# Autodesk Inventor assembly: Flywheel Axle Assembly v11
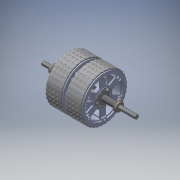
[picture p0: Inventor's stored thumbnail of the model, 180x180]
Saved by Autodesk Inventor 2018 (Build 220112000, 112)
## iProperties
Created: 2020-01-29
Part Number: Flywheel Axle Assembly v11
Document SubType Name: Assembly
Designer: s-2512711
Author: s-2512711
## Documents named in this file (10)
- \\studenthome\students\S-2512711\GitHub\2020CAD\New Gabriel Shooter\ACTUAL ASSEMBLY FILES\Flywheel Axle Assembly v11.iam
- \\studenthome\students\S-2512711\GitHub\2020CAD\New Gabriel Shooter\ACTUAL ASSEMBLY FILES\am-2986 FR8ZZ Hex Bearing v1.ipt
- \\studenthome\students\S-2512711\GitHub\2020CAD\New Gabriel Shooter\ACTUAL ASSEMBLY FILES\6_Traction_Tire_mounted_on_6_Traction_Wheel v1.iam
- \\studenthome\students\S-2512711\GitHub\2020CAD\New Gabriel Shooter\ACTUAL ASSEMBLY FILES\6_Traction_Tire_mounted_on_6_Traction_Wheel v1_1.iam
- \\studenthome\students\S-2512711\GitHub\2020CAD\New Gabriel Shooter\ACTUAL ASSEMBLY FILES\1_2_Hex_Bore_Aluminum_VersaHub_217-2592 v1.ipt
- \\studenthome\students\S-2512711\GitHub\2020CAD\New Gabriel Shooter\ACTUAL ASSEMBLY FILES\1_2_Acetal_Spacer_-_1_2_Hex_217-3261 v1.ipt
- \\studenthome\students\S-2512711\GitHub\2020CAD\New Gabriel Shooter\ACTUAL ASSEMBLY FILES\1_16_Acetal_Spacer_-_1_2_Hex_217-3257 v1.ipt
- \\studenthome\students\S-2512711\GitHub\2020CAD\New Gabriel Shooter\ACTUAL ASSEMBLY FILES\1_Acetal_Spacer_-_1_2_Hex_217-3263 v1.ipt
- \\studenthome\students\S-2512711\GitHub\2020CAD\New Gabriel Shooter\ACTUAL ASSEMBLY FILES\1_4_Acetal_Spacer_-_1_2_Hex_217-3259 v1.ipt
- \\studenthome\students\S-2512711\GitHub\2020CAD\New Gabriel Shooter\ACTUAL ASSEMBLY FILES\Flywheel Axle Assembly v11.ipt
## Components (18 placed, 8 different names)
1. am-2986 FR8ZZ Hex Bearing v1:1 — Mate:19, Mate:20, Mate:21
2. am-2986 FR8ZZ Hex Bearing v1:2 — Mate:1, Mate:2, Mate:3
3. 6_Traction_Tire_mounted_on_6_Traction_Wheel v1:1 [sub-assembly] — Mate:26, Mate:27, Mate:28, Mate:29, Mate:30, Mate:31
4. 6_Traction_Tire_mounted_on_6_Traction_Wheel v1:2 [sub-assembly] — Mate:10, Mate:11, Mate:12, Mate:13, Mate:14, Mate:15
5. 1_2_Hex_Bore_Aluminum_VersaHub_217-2592 v1:1 — Mate:25, Mate:26, Mate:27, Mate:28
6. 1_2_Hex_Bore_Aluminum_VersaHub_217-2592 v1:2 — Mate:29, Mate:30, Mate:31, Mate:32
7. 1_2_Hex_Bore_Aluminum_VersaHub_217-2592 v1:3 — Mate:13, Mate:14, Mate:15, Mate:18
8. 1_2_Hex_Bore_Aluminum_VersaHub_217-2592 v1:4 — Mate:7, Mate:8, Mate:9, Mate:10, Mate:11, Mate:12
9. 1_2_Acetal_Spacer_-_1_2_Hex_217-3261 v1:1 — Mate:16, Mate:17, Mate:18, Mate:32
10. 1_2_Acetal_Spacer_-_1_2_Hex_217-3261 v1:2 — Mate:23, Mate:24
11. 1_2_Acetal_Spacer_-_1_2_Hex_217-3261 v1:3 — Mate:5, Mate:6
12. 1_16_Acetal_Spacer_-_1_2_Hex_217-3257 v1:1 — Mate:3, Mate:4
13. 1_16_Acetal_Spacer_-_1_2_Hex_217-3257 v1:2 — Mate:21, Mate:22
14. 1_Acetal_Spacer_-_1_2_Hex_217-3263 v1:1 — Mate:6, Mate:7
15. 1_Acetal_Spacer_-_1_2_Hex_217-3263 v1:2 — Mate:24, Mate:25
16. 1_4_Acetal_Spacer_-_1_2_Hex_217-3259 v1:1 — Mate:22, Mate:23
17. 1_4_Acetal_Spacer_-_1_2_Hex_217-3259 v1:2 — Mate:4, Mate:5
18. Flywheel Axle Assembly v11 — Mate:1, Mate:2, Mate:8, Mate:9, Mate:16, Mate:17, Mate:19, Mate:20
## Relationships (32: Mate 32)
- Mate:1: am-2986 FR8ZZ Hex Bearing v1:2 ↔ Flywheel Axle Assembly v11
- Mate:2: am-2986 FR8ZZ Hex Bearing v1:2 ↔ Flywheel Axle Assembly v11
- Mate:3: am-2986 FR8ZZ Hex Bearing v1:2 ↔ 1_16_Acetal_Spacer_-_1_2_Hex_217-3257 v1:1
- Mate:4: 1_16_Acetal_Spacer_-_1_2_Hex_217-3257 v1:1 ↔ 1_4_Acetal_Spacer_-_1_2_Hex_217-3259 v1:2
- Mate:5: 1_2_Acetal_Spacer_-_1_2_Hex_217-3261 v1:3 ↔ 1_4_Acetal_Spacer_-_1_2_Hex_217-3259 v1:2
- Mate:6: 1_2_Acetal_Spacer_-_1_2_Hex_217-3261 v1:3 ↔ 1_Acetal_Spacer_-_1_2_Hex_217-3263 v1:1
- Mate:7: 1_2_Hex_Bore_Aluminum_VersaHub_217-2592 v1:4 ↔ 1_Acetal_Spacer_-_1_2_Hex_217-3263 v1:1
- Mate:8: 1_2_Hex_Bore_Aluminum_VersaHub_217-2592 v1:4 ↔ Flywheel Axle Assembly v11
- Mate:9: 1_2_Hex_Bore_Aluminum_VersaHub_217-2592 v1:4 ↔ Flywheel Axle Assembly v11
- Mate:10: 6_Traction_Tire_mounted_on_6_Traction_Wheel v1:2 ↔ 1_2_Hex_Bore_Aluminum_VersaHub_217-2592 v1:4
- Mate:11: 6_Traction_Tire_mounted_on_6_Traction_Wheel v1:2 ↔ 1_2_Hex_Bore_Aluminum_VersaHub_217-2592 v1:4
- Mate:12: 6_Traction_Tire_mounted_on_6_Traction_Wheel v1:2 ↔ 1_2_Hex_Bore_Aluminum_VersaHub_217-2592 v1:4
- Mate:13: 6_Traction_Tire_mounted_on_6_Traction_Wheel v1:2 ↔ 1_2_Hex_Bore_Aluminum_VersaHub_217-2592 v1:3
- Mate:14: 6_Traction_Tire_mounted_on_6_Traction_Wheel v1:2 ↔ 1_2_Hex_Bore_Aluminum_VersaHub_217-2592 v1:3
- Mate:15: 6_Traction_Tire_mounted_on_6_Traction_Wheel v1:2 ↔ 1_2_Hex_Bore_Aluminum_VersaHub_217-2592 v1:3
- Mate:16: 1_2_Acetal_Spacer_-_1_2_Hex_217-3261 v1:1 ↔ Flywheel Axle Assembly v11
- Mate:17: 1_2_Acetal_Spacer_-_1_2_Hex_217-3261 v1:1 ↔ Flywheel Axle Assembly v11
- Mate:18: 1_2_Hex_Bore_Aluminum_VersaHub_217-2592 v1:3 ↔ 1_2_Acetal_Spacer_-_1_2_Hex_217-3261 v1:1
- Mate:19: am-2986 FR8ZZ Hex Bearing v1:1 ↔ Flywheel Axle Assembly v11
- Mate:20: am-2986 FR8ZZ Hex Bearing v1:1 ↔ Flywheel Axle Assembly v11
- Mate:21: am-2986 FR8ZZ Hex Bearing v1:1 ↔ 1_16_Acetal_Spacer_-_1_2_Hex_217-3257 v1:2
- Mate:22: 1_16_Acetal_Spacer_-_1_2_Hex_217-3257 v1:2 ↔ 1_4_Acetal_Spacer_-_1_2_Hex_217-3259 v1:1
- Mate:23: 1_2_Acetal_Spacer_-_1_2_Hex_217-3261 v1:2 ↔ 1_4_Acetal_Spacer_-_1_2_Hex_217-3259 v1:1
- Mate:24: 1_2_Acetal_Spacer_-_1_2_Hex_217-3261 v1:2 ↔ 1_Acetal_Spacer_-_1_2_Hex_217-3263 v1:2
- Mate:25: 1_2_Hex_Bore_Aluminum_VersaHub_217-2592 v1:1 ↔ 1_Acetal_Spacer_-_1_2_Hex_217-3263 v1:2
- Mate:26: 6_Traction_Tire_mounted_on_6_Traction_Wheel v1:1 ↔ 1_2_Hex_Bore_Aluminum_VersaHub_217-2592 v1:1
- Mate:27: 6_Traction_Tire_mounted_on_6_Traction_Wheel v1:1 ↔ 1_2_Hex_Bore_Aluminum_VersaHub_217-2592 v1:1
- Mate:28: 6_Traction_Tire_mounted_on_6_Traction_Wheel v1:1 ↔ 1_2_Hex_Bore_Aluminum_VersaHub_217-2592 v1:1
- Mate:29: 6_Traction_Tire_mounted_on_6_Traction_Wheel v1:1 ↔ 1_2_Hex_Bore_Aluminum_VersaHub_217-2592 v1:2
- Mate:30: 6_Traction_Tire_mounted_on_6_Traction_Wheel v1:1 ↔ 1_2_Hex_Bore_Aluminum_VersaHub_217-2592 v1:2
- Mate:31: 6_Traction_Tire_mounted_on_6_Traction_Wheel v1:1 ↔ 1_2_Hex_Bore_Aluminum_VersaHub_217-2592 v1:2
- Mate:32: 1_2_Hex_Bore_Aluminum_VersaHub_217-2592 v1:2 ↔ 1_2_Acetal_Spacer_-_1_2_Hex_217-3261 v1:1
